# Autodesk Inventor assembly: z_shaft
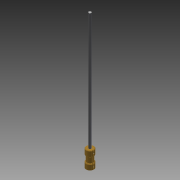
[picture p0: Inventor's stored thumbnail of the model, 180x180]
Saved by Autodesk Inventor 2013 (Build 170138000, 138)
## iProperties
Created: 2015-02-20
Part Number: z_shaft
Document SubType Name: Assembly
Designer: Noa Izumi
Author: Noa Izumi
## Documents named in this file (3)
- C:\reprap\TinyBoy_v3_20150220\z_shaft.iam
- C:\reprap\TinyBoy_v3_20150220\coupler_0305.ipt
- C:\reprap\TinyBoy_v3_20150220\thread_M3_150.ipt
## Components (2 placed, 2 different names)
1. coupler_0305:1 — 插入:1
2. thread_M3_150:1 — 插入:1
## Relationships (1: Insert 1)
- 插入:1 [Insert]: coupler_0305:1 ↔ thread_M3_150:1
